# Autodesk Inventor assembly: Shoulder_CrossRollerBearingUnit
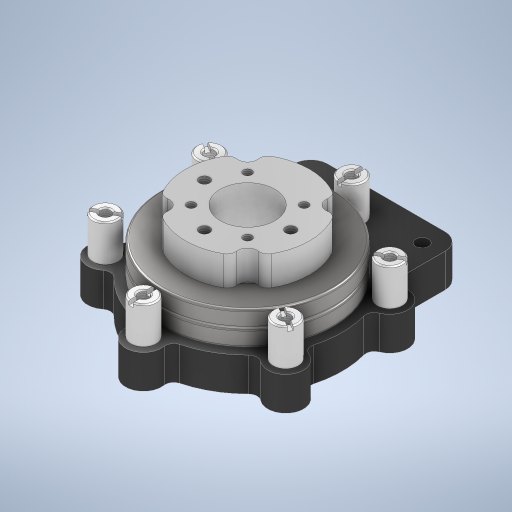
[picture p0: Inventor's stored thumbnail of the model, 512x512]
Saved by Autodesk Inventor 2024.2 (Build 282272000, 272)
## iProperties
Created: 2024-01-04
Part Number: Shoulder_CrossRollerBearingUnit
Document SubType Name: Assembly
Designer: Masato Kubotera
Mass: 101.427 g
Surface Area: 162.729 cm^2
Volume: 22.4446 cm^3
Density: 4.51898 g/cm^3
Author: Masato Kubotera
## Documents named in this file (9)
- C:\Users\masato\OneDrive - Chiba Institute of Technology\CIT Brains\RoboCup2024\Mechanic\SUSTAINA-OP2\NativeFiles\Boby\CommonDesignedComponents\CrossRollerBearingUnit\Shoulder_CrossRollerBearingUnit.iam
- C:\Users\masato\OneDrive - Chiba Institute of Technology\CIT Brains\RoboCup2024\Mechanic\SUSTAINA-OP2\NativeFiles\Boby\COTS\Bearings\RB2508UUC0.ipt
- C:\Users\masato\OneDrive - Chiba Institute of Technology\CIT Brains\RoboCup2024\Mechanic\SUSTAINA-OP2\NativeFiles\Boby\CommonDesignedComponents\CrossRollerBearingUnit\CrossRollerBearingInnerFlange.ipt
- C:\Users\masato\OneDrive - Chiba Institute of Technology\CIT Brains\RoboCup2024\Mechanic\SUSTAINA-OP2\NativeFiles\Boby\CommonDesignedComponents\CrossRollerBearingUnit\CrossRollerBearingInnerSupportStand.ipt
- C:\Users\masato\OneDrive - Chiba Institute of Technology\CIT Brains\RoboCup2024\Mechanic\SUSTAINA-OP2\NativeFiles\Boby\CommonDesignedComponents\CrossRollerBearingUnit\Shoulder_CrossRollerBearingOuterFlange.ipt
- C:\Users\masato\OneDrive - Chiba Institute of Technology\CIT Brains\RoboCup2024\Mechanic\SUSTAINA-OP2\NativeFiles\Boby\COTS\Spacers\ARU-309S.ipt
- C:\Users\masato\OneDrive - Chiba Institute of Technology\CIT Brains\RoboCup2024\Mechanic\SUSTAINA-OP2\NativeFiles\Boby\COTS\Spacers\BRU-309S.ipt
- C:\Users\masato\OneDrive - Chiba Institute of Technology\CIT Brains\RoboCup2024\Mechanic\SUSTAINA-OP2\NativeFiles\Boby\COTS\Screws\ScrewsWithShoulder\LMSBP4-10.ipt
- C:\Users\masato\OneDrive - Chiba Institute of Technology\CIT Brains\RoboCup2024\Mechanic\SUSTAINA-OP2\NativeFiles\Boby\COTS\Screws\CapScrew\UC-0306.ipt
## Components (15 placed, 8 different names)
1. Shoulder_CrossRollerBearingOuterFlange:1 — Insert:12, Angle:9, Insert:13, Insert:14, Insert:15
2. CrossRollerBearingInnerFlange:1 — Insert:7, Angle:4, Insert:16
3. CrossRollerBearingInnerSupportStand:1 — Insert:11, Angle:8
4. UC-0306:1 — Insert:15
5. ARU-309S:1 — Insert:14, Angle:10
6. RB2508UUC0:1 — Flush:4, Flush:5, Insert:7, Insert:11, Insert:12
7. BRU-309S:1 — Insert:13, Angle:11
8. BRU-309S:2
9. BRU-309S:3
10. BRU-309S:4
11. BRU-309S:5
12. LMSBP4-10:1 — Insert:16
13. LMSBP4-10:2
14. LMSBP4-10:3
15. LMSBP4-10:4
## Component patterns: (5 elements, first: BRU-309S:1), (4 elements, first: LMSBP4-10:1)
## Relationships (14: Insert 7, Angle 5, Flush 2)
- Flush:4: RB2508UUC0:1
- Flush:5: RB2508UUC0:1
- Insert:7: CrossRollerBearingInnerFlange:1 ↔ RB2508UUC0:1
- Angle:4 (0 deg): CrossRollerBearingInnerFlange:1
- Insert:11: CrossRollerBearingInnerSupportStand:1 ↔ RB2508UUC0:1
- Angle:8 (0 deg): CrossRollerBearingInnerSupportStand:1
- Insert:12: Shoulder_CrossRollerBearingOuterFlange:1 ↔ RB2508UUC0:1
- Angle:9 (0 deg): Shoulder_CrossRollerBearingOuterFlange:1
- Insert:13: Shoulder_CrossRollerBearingOuterFlange:1 ↔ BRU-309S:1
- Insert:14: Shoulder_CrossRollerBearingOuterFlange:1 ↔ ARU-309S:1
- Angle:10 (0 deg): ARU-309S:1
- Angle:11 (60 deg): BRU-309S:1
- Insert:15: Shoulder_CrossRollerBearingOuterFlange:1 ↔ UC-0306:1
- Insert:16: CrossRollerBearingInnerFlange:1 ↔ LMSBP4-10:1
